# Autodesk Inventor assembly: Inner_Components
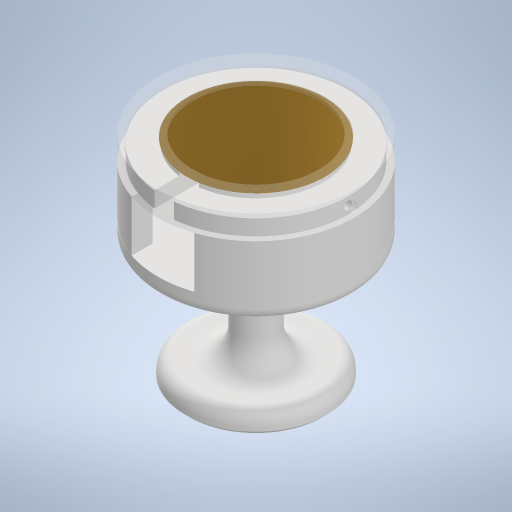
[picture p0: Inventor's stored thumbnail of the model, 512x512]
Saved by Autodesk Inventor 2023 (Build 270158000, 158)
## iProperties
Created: 2023-02-27
Part Number: Inner_Components
Document SubType Name: Assembly
Designer: maste
Author: maste
## Documents named in this file (5)
- C:\Users\maste\Documents\GitHub\Remote-Stethoscope\3D_models\ThonkLabs 1ne\SurfaceContact\Inner_Components.iam
- C:\Users\maste\Documents\GitHub\Remote-Stethoscope\3D_models\ThonkLabs 1ne\SurfaceContact\PiezoMount.ipt
- C:\Users\maste\Documents\GitHub\Remote-Stethoscope\3D_models\ThonkLabs 1ne\SurfaceContact\Piezo.ipt
- C:\Users\maste\Documents\GitHub\Remote-Stethoscope\3D_models\ThonkLabs 1ne\SurfaceContact\Diaphragm_lock.ipt
- C:\Users\maste\Documents\GitHub\Remote-Stethoscope\3D_models\ThonkLabs 1ne\SurfaceContact\holding_socket.ipt
## Components (4 placed, 4 different names)
1. PiezoMount:1 — Mate:2, Mate:7, Mate:8, Mate:9, Mate:10, Mate:11, Mate:12
2. Piezo:1 — Mate:2, Mate:12, Mate:13
3. Diaphragm_lock:1 — Mate:11, Mate:13
4. holding_socket:1 — Mate:7, Mate:8, Mate:9, Mate:10
## Relationships (8: Mate 8)
- Mate:2: PiezoMount:1 ↔ Piezo:1
- Mate:7: PiezoMount:1 ↔ holding_socket:1
- Mate:8: PiezoMount:1 ↔ holding_socket:1
- Mate:9: PiezoMount:1 ↔ holding_socket:1
- Mate:10: PiezoMount:1 ↔ holding_socket:1
- Mate:11: PiezoMount:1 ↔ Diaphragm_lock:1
- Mate:12: PiezoMount:1 ↔ Piezo:1
- Mate:13: Piezo:1 ↔ Diaphragm_lock:1
